# Autodesk Inventor assembly: DO-214AB (SMC) установка
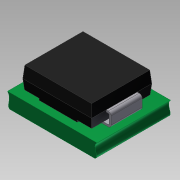
[picture p0: Inventor's stored thumbnail of the model, 180x180]
Saved by Autodesk Inventor 2011 (Build 150239000, 239)
## iProperties
Created: 2011-01-13
Part Number: DO-214AB (SMC) установка
Document SubType Name: Assembly
Designer: abbath
Author: abbath
## Documents named in this file (3)
- D:\Abbath\Work\11.2\Сумматор light\КД\RSXX к сумматору\Установка элементов\DO-214AB (SMC) установка.iam
- D:\Abbath\Work\11.2\Сумматор light\КД\RSXX к сумматору\Установка элементов\DO-214AB (SMC).ipt
- D:\Abbath\Work\11.2\Сумматор light\КД\RSXX к сумматору\Установка элементов\DO-214AB (SMC) плата.ipt
## Components (2 placed, 2 different names)
1. DO-214AB (SMC):1 — Заподлицо:1
2. DO-214AB (SMC) плата:1 — Заподлицо:1
## Relationships (1: Flush 1)
- Заподлицо:1 [Flush]: DO-214AB (SMC):1 ↔ DO-214AB (SMC) плата:1
